# Autodesk Inventor assembly: Full payload assembly mk 2
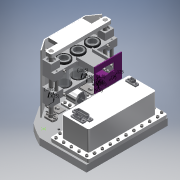
[picture p0: Inventor's stored thumbnail of the model, 180x180]
Saved by Autodesk Inventor 2017 (Build 210142000, 142)
## iProperties
Created: 2016-12-06
Part Number: Full payload assembly mk 2
Document SubType Name: Assembly
Designer: qupec
Mass: 1513.48 g
Surface Area: 2866.97 cm^2
Volume: 582.995 cm^3
Density: 2.59604 g/cm^3
Author: qupec
## Documents named in this file (37)
- D:\UMD Near Space\star\CAD\Mechanical\Full payload assembly mk 2.iam
- D:\UMD Near Space\star\CAD\Mechanical\Subsystems\Slide Rods\Slide rod assembly.iam
- D:\UMD Near Space\star\CAD\Mechanical\Subsystems\Test Tube Rack\Test tube rack.iam
- D:\UMD Near Space\star\CAD\Mechanical\Electonics\STARduino and Pi assembly.iam
- D:\UMD Near Space\star\CAD\Mechanical\Subsystems\Video Capture\Pi Cam and Cable assembly.iam
- D:\UMD Near Space\star\CAD\Mechanical\Electonics\Ribbon Cable Connector-02.ipt
- D:\UMD Near Space\star\CAD\Mechanical\Full payload assembly\AIP\Cable and Harness\Full payload assembly.Harness2.iam
- C:\Users\qupec\Documents\Inventor\Content Center Files\R2017\en-US\U UNC 2603(1)\Unbrako - 4 x 1 - 48 - 1 - Unbrako.ipt
- D:\UMD Near Space\star\CAD\Mechanical\Subsystems\ShakerCAD\ShakerAssembly.iam
- D:\UMD Near Space\star\CAD\Mechanical\Base Plate Mk 2.ipt
- D:\UMD Near Space\star\CAD\Mechanical\Electonics\Electronics Box.ipt
- D:\UMD Near Space\star\CAD\Mechanical\Electonics\Sensor Board.ipt
- D:\UMD Near Space\star\CAD\Mechanical\Electonics\9pin female connector.ipt
- D:\UMD Near Space\star\CAD\Mechanical\Electonics\31pin female connector.ipt
- D:\UMD Near Space\star\CAD\Mechanical\Electonics\15pin female connector.ipt
- C:\Users\qupec\Documents\Inventor\Content Center Files\R2017\en-US\ANSI B18.3(05)\ANSI B18.3 - 4-40 UNC - 0.625(31).ipt
- C:\Users\qupec\Documents\Inventor\Content Center Files\R2017\en-US\ANSI B18.3(05)\ANSI B18.3 - 4-40 UNC - 0.5(31).ipt
- D:\UMD Near Space\star\CAD\Mechanical\Subsystems\Video Capture\LED 5mm.ipt
- C:\Users\qupec\Documents\Inventor\Content Center Files\R2017\en-US\ANSI B18.3(05)\ANSI B18.3 - 4-40 UNC - 0.1875(31).ipt
- D:\UMD Near Space\star\CAD\Mechanical\solar sheild.ipt
- D:\UMD Near Space\star\CAD\Mechanical\Emergency Battery.ipt
- C:\Users\qupec\Documents\Inventor\Content Center Files\R2017\en-US\ANSI B18.3(05)\ANSI B18.3 - 4-40 UNC - 0.75(31).ipt
- D:\UMD Near Space\star\CAD\Mechanical\1556A410_BRACKET.ipt
- D:\UMD Near Space\star\CAD\Mechanical\94518A210_MIL SPEC FLAT-HEAD SOCKET CAP SCREW.ipt
- D:\UMD Near Space\star\CAD\Mechanical\98019A314_MIL SPEC. 300 SERIES SS FLAT WASHER.ipt
- D:\UMD Near Space\star\CAD\Mechanical\Subsystems\Full payload assembly mk 2\AIP\FEA\c3occb59c.fins
- D:\UMD Near Space\star\CAD\Mechanical\Subsystems\Full payload assembly mk 2\AIP\FEA\c3occb5b4.fsat
- D:\UMD Near Space\star\CAD\Mechanical\Subsystems\Full payload assembly mk 2\AIP\FEA\c3occb5b4.ftes
- D:\UMD Near Space\star\CAD\Mechanical\Subsystems\Full payload assembly mk 2\AIP\FEA\c3occb5b4.fwiz
- D:\UMD Near Space\star\CAD\Mechanical\Subsystems\Full payload assembly mk 2\AIP\FEA\c3occb5c0.fins
- D:\UMD Near Space\star\CAD\Mechanical\Subsystems\Full payload assembly mk 2\AIP\FEA\c3occb5c0.fsat
- D:\UMD Near Space\star\CAD\Mechanical\Subsystems\Full payload assembly mk 2\AIP\FEA\c3occb5c0.ftes
- D:\UMD Near Space\star\CAD\Mechanical\Subsystems\Full payload assembly mk 2\AIP\FEA\c3occb5c0.fwiz
- D:\UMD Near Space\star\CAD\Mechanical\Subsystems\Full payload assembly mk 2\AIP\FEA\c3occb60w.fmsh
- D:\UMD Near Space\star\CAD\Mechanical\Subsystems\Full payload assembly mk 2\AIP\FEA\c3occb60x.fres
- D:\UMD Near Space\star\CAD\Mechanical\Subsystems\Full payload assembly mk 2\AIP\FEA\c3occb6sg.fmsh
- D:\UMD Near Space\star\CAD\Mechanical\Subsystems\Full payload assembly mk 2\AIP\FEA\c3occb6sh.fres
## Components (66 placed, 24 different names)
1. Slide rod assembly:1 [sub-assembly] — Mate:119, Mate:120, Mate:121, Mate:278, Mate:280, Mate:282, Mate:284, Mate:286, Mate:288, Mate:290, Mate:292, Mate:294, Mate:296, Flush:47, Mate:382
2. Test tube rack:1 [sub-assembly] — Mate:56, Flush:19, Flush:20, Mate:113, Mate:114, Mate:119, Mate:120, Flush:45
3. Pi Cam and Cable assembly:1 [sub-assembly] — Mate:56, Flush:19, Flush:20, Mate:169, Mate:171, Insert:1, Mate:299, Mate:300, Mate:302, Mate:303, Mate:304
4. Ribbon Cable Connector-02:1 — Mate:80, Flush:24, Flush:25
5. Harness2 [sub-assembly]
6. STARduino and Pi assembly:1 [sub-assembly] — Mate:80, Flush:24, Flush:25, Mate:122, Flush:41, Flush:42, Flush:46
7. ShakerAssembly:1 [sub-assembly] — Mate:113, Mate:114, Flush:26, Mate:123, Angle:2
8. Base Plate Mk 2:1 — Mate:121, Flush:26, Mate:122, Mate:123, Mate:124, Flush:29, Flush:32, Mate:163, Flush:33, Flush:40, Mate:277, Mate:279, Mate:281, Mate:283, Mate:285, Mate:287, Mate:289, Mate:291, Mate:293, Mate:295, Mate:307, Mate:309, Mate:311, Mate:313, Mate:315, Mate:317, Mate:319, Mate:321, Mate:323, Mate:325, Mate:327, Mate:329, Mate:331, Mate:333, Mate:335, Mate:337, Mate:339, Mate:341, Mate:343, Mate:345, Mate:347, Mate:349, Mate:351, Mate:353, Mate:355, Mate:357, Mate:359, Mate:361, Flush:45, Mate:373, Mate:374, Mate:375, Mate:376, Mate:377
9. Sensor Board:1 — Angle:1, Mate:303, Mate:304, Mate:305, Mate:306
10. 31pin female connector:1 — Flush:34, Flush:35, Mate:164
11. 15pin female connector:1 — Mate:165, Flush:43, Flush:44
12. 9pin female connector:1 — Flush:38, Flush:39, Mate:166
13. Electronics Box:1 — Mate:163, Flush:33, Flush:34, Flush:35, Mate:164, Flush:38, Flush:39, Mate:165, Mate:166, Flush:40, Flush:41, Flush:42, Flush:43, Flush:44, Mate:308, Mate:310, Mate:312, Mate:314, Mate:316, Mate:318, Mate:320, Mate:322, Mate:324, Mate:326, Mate:328, Mate:330, Mate:332, Mate:334, Mate:336, Mate:338, Mate:340, Mate:342, Mate:344, Mate:346, Mate:348, Mate:350, Mate:352, Mate:354, Mate:356, Mate:358, Mate:360, Mate:362, Mate:372
14. Hexagon Socket Head Cap Screw - Inch No. 4 - 40 UNC - 1/2:1
15. Hexagon Socket Head Cap Screw - Inch No. 4 - 40 UNC - 1/2:2
16. Unbrako UNC Hex Socket Cap - Inch 4 x 1 - Unbrako:13 — Mate:169, Mate:171
17. Hexagon Socket Head Cap Screw - Inch No. 4 - 40 UNC - 5/8:1 — Mate:277, Mate:278
18. Hexagon Socket Head Cap Screw - Inch No. 4 - 40 UNC - 5/8:2 — Mate:279, Mate:280
19. Hexagon Socket Head Cap Screw - Inch No. 4 - 40 UNC - 5/8:3 — Mate:281, Mate:282
20. Hexagon Socket Head Cap Screw - Inch No. 4 - 40 UNC - 5/8:4 — Mate:283, Mate:284
21. Hexagon Socket Head Cap Screw - Inch No. 4 - 40 UNC - 5/8:5 — Mate:285, Mate:286
22. Hexagon Socket Head Cap Screw - Inch No. 4 - 40 UNC - 5/8:6 — Mate:287, Mate:288
23. Hexagon Socket Head Cap Screw - Inch No. 4 - 40 UNC - 5/8:7 — Mate:289, Mate:290
24. Hexagon Socket Head Cap Screw - Inch No. 4 - 40 UNC - 5/8:8 — Mate:291, Mate:292
25. Hexagon Socket Head Cap Screw - Inch No. 4 - 40 UNC - 5/8:9 — Mate:293, Mate:294
26. Hexagon Socket Head Cap Screw - Inch No. 4 - 40 UNC - 5/8:10 — Mate:295, Mate:296
27. Hexagon Socket Head Cap Screw - Inch No. 4 - 40 UNC - 5/8:11 — Insert:1
28. LED 5mm:1 — Mate:299, Mate:301, Mate:302, Mate:305
29. LED 5mm:2 — Mate:300, Mate:301, Mate:306
30. Hexagon Socket Head Cap Screw - Inch No. 4 - 40 UNC - 3/4:1 — Mate:307, Mate:308
31. Hexagon Socket Head Cap Screw - Inch No. 4 - 40 UNC - 3/4:2 — Mate:309, Mate:310
32. Hexagon Socket Head Cap Screw - Inch No. 4 - 40 UNC - 3/4:3 — Mate:311, Mate:312
33. Hexagon Socket Head Cap Screw - Inch No. 4 - 40 UNC - 3/4:4 — Mate:313, Mate:314
34. Hexagon Socket Head Cap Screw - Inch No. 4 - 40 UNC - 3/4:5 — Mate:315, Mate:316
35. Hexagon Socket Head Cap Screw - Inch No. 4 - 40 UNC - 3/16:6 — Mate:317, Mate:318
36. Hexagon Socket Head Cap Screw - Inch No. 4 - 40 UNC - 3/16:7 — Mate:319, Mate:320
37. Hexagon Socket Head Cap Screw - Inch No. 4 - 40 UNC - 3/16:8 — Mate:321, Mate:322
38. Hexagon Socket Head Cap Screw - Inch No. 4 - 40 UNC - 3/16:9 — Mate:323, Mate:324
39. Hexagon Socket Head Cap Screw - Inch No. 4 - 40 UNC - 3/16:10 — Mate:325, Mate:326
40. Hexagon Socket Head Cap Screw - Inch No. 4 - 40 UNC - 3/16:11 — Mate:327, Mate:328
41. Hexagon Socket Head Cap Screw - Inch No. 4 - 40 UNC - 3/16:12 — Mate:329, Mate:330
42. Hexagon Socket Head Cap Screw - Inch No. 4 - 40 UNC - 3/16:13 — Mate:331, Mate:332
43. Hexagon Socket Head Cap Screw - Inch No. 4 - 40 UNC - 3/16:14 — Mate:333, Mate:334
44. Hexagon Socket Head Cap Screw - Inch No. 4 - 40 UNC - 3/16:15 — Mate:335, Mate:336
45. Hexagon Socket Head Cap Screw - Inch No. 4 - 40 UNC - 3/16:16 — Mate:337, Mate:338
46. Hexagon Socket Head Cap Screw - Inch No. 4 - 40 UNC - 3/16:17 — Mate:339, Mate:340
47. Hexagon Socket Head Cap Screw - Inch No. 4 - 40 UNC - 1/2:3 — Mate:341, Mate:342
48. Hexagon Socket Head Cap Screw - Inch No. 4 - 40 UNC - 3/16:19 — Mate:343, Mate:344
49. Hexagon Socket Head Cap Screw - Inch No. 4 - 40 UNC - 3/16:20 — Mate:345, Mate:346
50. Hexagon Socket Head Cap Screw - Inch No. 4 - 40 UNC - 3/16:21 — Mate:347, Mate:348
51. Hexagon Socket Head Cap Screw - Inch No. 4 - 40 UNC - 3/16:22 — Mate:349, Mate:350
52. Hexagon Socket Head Cap Screw - Inch No. 4 - 40 UNC - 3/16:23 — Mate:351, Mate:352
53. Hexagon Socket Head Cap Screw - Inch No. 4 - 40 UNC - 3/16:24 — Mate:353, Mate:354
54. Hexagon Socket Head Cap Screw - Inch No. 4 - 40 UNC - 3/16:25 — Mate:355, Mate:356
55. Hexagon Socket Head Cap Screw - Inch No. 4 - 40 UNC - 3/16:26 — Mate:357, Mate:358
56. Hexagon Socket Head Cap Screw - Inch No. 4 - 40 UNC - 3/16:27 — Mate:359, Mate:360
57. Hexagon Socket Head Cap Screw - Inch No. 4 - 40 UNC - 3/16:28 — Mate:361, Mate:362
58. solar sheild:1 — Mate:378, Mate:379, Mate:380, Flush:47, Mate:381, Mate:382
59. Emergency Battery:1 — Mate:372, Mate:373, Flush:46
60. 1556A410_BRACKET:1 — Mate:375, Mate:377, Angle:3, Mate:379, Mate:381, Mate:384, Mate:387, Mate:388
61. 1556A410_BRACKET:2 — Mate:374, Mate:376, Angle:2, Angle:3, Mate:378, Mate:380, Mate:383, Mate:386
62. 94518A210_MIL SPEC FLAT-HEAD SOCKET CAP SCREW:1 — Mate:384, Flush:48
63. 94518A210_MIL SPEC FLAT-HEAD SOCKET CAP SCREW:2 — Mate:383, Flush:48, Mate:385
64. 98019A314_MIL SPEC. 300 SERIES SS FLAT WASHER:1
65. 98019A314_MIL SPEC. 300 SERIES SS FLAT WASHER:2 — Mate:385, Mate:386
66. 98019A314_MIL SPEC. 300 SERIES SS FLAT WASHER:3 — Mate:387, Mate:388
## Relationships (146: Mate 121, Flush 21, Angle 3, Insert 1)
- Mate:56: Test tube rack:1 ↔ Pi Cam and Cable assembly:1
- Flush:19: Test tube rack:1 ↔ Pi Cam and Cable assembly:1
- Flush:20: Test tube rack:1 ↔ Pi Cam and Cable assembly:1
- Mate:80: Ribbon Cable Connector-02:1 ↔ STARduino and Pi assembly:1
- Flush:24 (-7 mm): Ribbon Cable Connector-02:1 ↔ STARduino and Pi assembly:1
- Flush:25: Ribbon Cable Connector-02:1 ↔ STARduino and Pi assembly:1
- Mate:113: Test tube rack:1 ↔ ShakerAssembly:1
- Mate:114: Test tube rack:1 ↔ ShakerAssembly:1
- Mate:119: Slide rod assembly:1 ↔ Test tube rack:1
- Mate:120: Slide rod assembly:1 ↔ Test tube rack:1
- Mate:121: Slide rod assembly:1 ↔ Base Plate Mk 2:1
- Flush:26 (6.604 mm): ShakerAssembly:1 ↔ Base Plate Mk 2:1
- Mate:122: STARduino and Pi assembly:1 ↔ Base Plate Mk 2:1
- Mate:123: ShakerAssembly:1 ↔ Base Plate Mk 2:1
- Mate:124: Base Plate Mk 2:1
- Flush:29: Base Plate Mk 2:1
- Flush:32: Base Plate Mk 2:1
- Angle:1 (0 deg): Sensor Board:1
- Mate:163: Base Plate Mk 2:1 ↔ Electronics Box:1
- Flush:33: Base Plate Mk 2:1 ↔ Electronics Box:1
- Flush:34 (12.7 mm): 31pin female connector:1 ↔ Electronics Box:1
- Flush:35 (6.35 mm): 31pin female connector:1 ↔ Electronics Box:1
- Mate:164: 31pin female connector:1 ↔ Electronics Box:1
- Flush:38 (6.35 mm): 9pin female connector:1 ↔ Electronics Box:1
- Flush:39 (-6.35 mm): 9pin female connector:1 ↔ Electronics Box:1
- Mate:165: 15pin female connector:1 ↔ Electronics Box:1
- Mate:166: 9pin female connector:1 ↔ Electronics Box:1
- Flush:40: Base Plate Mk 2:1 ↔ Electronics Box:1
- Flush:41 (3.175 mm): STARduino and Pi assembly:1 ↔ Electronics Box:1
- Flush:42: STARduino and Pi assembly:1 ↔ Electronics Box:1
- Flush:43 (3.81 mm): 15pin female connector:1 ↔ Electronics Box:1
- Flush:44 (12.7 mm): 15pin female connector:1 ↔ Electronics Box:1
- [Mate]: Pi Cam and Cable assembly:1 ↔ Hexagon Socket Head Cap Screw - Inch No. 4 - 40 UNC - 1/2:1
- [Mate]: Pi Cam and Cable assembly:1 ↔ Hexagon Socket Head Cap Screw - Inch No. 4 - 40 UNC - 1/2:2
- Mate:169: Pi Cam and Cable assembly:1 ↔ Unbrako UNC Hex Socket Cap - Inch 4 x 1 - Unbrako:13
- [Mate]: Pi Cam and Cable assembly:1 ↔ Hexagon Socket Head Cap Screw - Inch No. 4 - 40 UNC - 1/2:2
- Mate:171: Pi Cam and Cable assembly:1 ↔ Unbrako UNC Hex Socket Cap - Inch 4 x 1 - Unbrako:13
- [Mate]: Pi Cam and Cable assembly:1 ↔ Hexagon Socket Head Cap Screw - Inch No. 4 - 40 UNC - 1/2:1
- Mate:277: Base Plate Mk 2:1 ↔ Hexagon Socket Head Cap Screw - Inch No. 4 - 40 UNC - 5/8:1
- Mate:278: Slide rod assembly:1 ↔ Hexagon Socket Head Cap Screw - Inch No. 4 - 40 UNC - 5/8:1
- Mate:279: Base Plate Mk 2:1 ↔ Hexagon Socket Head Cap Screw - Inch No. 4 - 40 UNC - 5/8:2
- Mate:280: Slide rod assembly:1 ↔ Hexagon Socket Head Cap Screw - Inch No. 4 - 40 UNC - 5/8:2
- Mate:281: Base Plate Mk 2:1 ↔ Hexagon Socket Head Cap Screw - Inch No. 4 - 40 UNC - 5/8:3
- Mate:282: Slide rod assembly:1 ↔ Hexagon Socket Head Cap Screw - Inch No. 4 - 40 UNC - 5/8:3
- Mate:283: Base Plate Mk 2:1 ↔ Hexagon Socket Head Cap Screw - Inch No. 4 - 40 UNC - 5/8:4
- Mate:284: Slide rod assembly:1 ↔ Hexagon Socket Head Cap Screw - Inch No. 4 - 40 UNC - 5/8:4
- Mate:285: Base Plate Mk 2:1 ↔ Hexagon Socket Head Cap Screw - Inch No. 4 - 40 UNC - 5/8:5
- Mate:286: Slide rod assembly:1 ↔ Hexagon Socket Head Cap Screw - Inch No. 4 - 40 UNC - 5/8:5
- Mate:287: Base Plate Mk 2:1 ↔ Hexagon Socket Head Cap Screw - Inch No. 4 - 40 UNC - 5/8:6
- Mate:288: Slide rod assembly:1 ↔ Hexagon Socket Head Cap Screw - Inch No. 4 - 40 UNC - 5/8:6
- Mate:289: Base Plate Mk 2:1 ↔ Hexagon Socket Head Cap Screw - Inch No. 4 - 40 UNC - 5/8:7
- Mate:290: Slide rod assembly:1 ↔ Hexagon Socket Head Cap Screw - Inch No. 4 - 40 UNC - 5/8:7
- Mate:291: Base Plate Mk 2:1 ↔ Hexagon Socket Head Cap Screw - Inch No. 4 - 40 UNC - 5/8:8
- Mate:292: Slide rod assembly:1 ↔ Hexagon Socket Head Cap Screw - Inch No. 4 - 40 UNC - 5/8:8
- Mate:293: Base Plate Mk 2:1 ↔ Hexagon Socket Head Cap Screw - Inch No. 4 - 40 UNC - 5/8:9
- Mate:294: Slide rod assembly:1 ↔ Hexagon Socket Head Cap Screw - Inch No. 4 - 40 UNC - 5/8:9
- Mate:295: Base Plate Mk 2:1 ↔ Hexagon Socket Head Cap Screw - Inch No. 4 - 40 UNC - 5/8:10
- Mate:296: Slide rod assembly:1 ↔ Hexagon Socket Head Cap Screw - Inch No. 4 - 40 UNC - 5/8:10
- Insert:1: Pi Cam and Cable assembly:1 ↔ Hexagon Socket Head Cap Screw - Inch No. 4 - 40 UNC - 5/8:11
- Mate:299: Pi Cam and Cable assembly:1 ↔ LED 5mm:1
- Mate:300: Pi Cam and Cable assembly:1 ↔ LED 5mm:2
- Mate:301: LED 5mm:1 ↔ LED 5mm:2
- Mate:302: Pi Cam and Cable assembly:1 ↔ LED 5mm:1
- Mate:303: Pi Cam and Cable assembly:1 ↔ Sensor Board:1
- Mate:304: Pi Cam and Cable assembly:1 ↔ Sensor Board:1
- Mate:305: Sensor Board:1 ↔ LED 5mm:1
- Mate:306: Sensor Board:1 ↔ LED 5mm:2
- Mate:307: Base Plate Mk 2:1 ↔ Hexagon Socket Head Cap Screw - Inch No. 4 - 40 UNC - 3/4:1
- Mate:308: Electronics Box:1 ↔ Hexagon Socket Head Cap Screw - Inch No. 4 - 40 UNC - 3/4:1
- Mate:309: Base Plate Mk 2:1 ↔ Hexagon Socket Head Cap Screw - Inch No. 4 - 40 UNC - 3/4:2
- Mate:310: Electronics Box:1 ↔ Hexagon Socket Head Cap Screw - Inch No. 4 - 40 UNC - 3/4:2
- Mate:311: Base Plate Mk 2:1 ↔ Hexagon Socket Head Cap Screw - Inch No. 4 - 40 UNC - 3/4:3
- Mate:312: Electronics Box:1 ↔ Hexagon Socket Head Cap Screw - Inch No. 4 - 40 UNC - 3/4:3
- Mate:313: Base Plate Mk 2:1 ↔ Hexagon Socket Head Cap Screw - Inch No. 4 - 40 UNC - 3/4:4
- Mate:314: Electronics Box:1 ↔ Hexagon Socket Head Cap Screw - Inch No. 4 - 40 UNC - 3/4:4
- Mate:315: Base Plate Mk 2:1 ↔ Hexagon Socket Head Cap Screw - Inch No. 4 - 40 UNC - 3/4:5
- Mate:316: Electronics Box:1 ↔ Hexagon Socket Head Cap Screw - Inch No. 4 - 40 UNC - 3/4:5
- Mate:317: Base Plate Mk 2:1 ↔ Hexagon Socket Head Cap Screw - Inch No. 4 - 40 UNC - 3/16:6
- Mate:318: Electronics Box:1 ↔ Hexagon Socket Head Cap Screw - Inch No. 4 - 40 UNC - 3/16:6
- Mate:319: Base Plate Mk 2:1 ↔ Hexagon Socket Head Cap Screw - Inch No. 4 - 40 UNC - 3/16:7
- Mate:320: Electronics Box:1 ↔ Hexagon Socket Head Cap Screw - Inch No. 4 - 40 UNC - 3/16:7
- Mate:321: Base Plate Mk 2:1 ↔ Hexagon Socket Head Cap Screw - Inch No. 4 - 40 UNC - 3/16:8
- Mate:322: Electronics Box:1 ↔ Hexagon Socket Head Cap Screw - Inch No. 4 - 40 UNC - 3/16:8
- Mate:323: Base Plate Mk 2:1 ↔ Hexagon Socket Head Cap Screw - Inch No. 4 - 40 UNC - 3/16:9
- Mate:324: Electronics Box:1 ↔ Hexagon Socket Head Cap Screw - Inch No. 4 - 40 UNC - 3/16:9
- Mate:325: Base Plate Mk 2:1 ↔ Hexagon Socket Head Cap Screw - Inch No. 4 - 40 UNC - 3/16:10
- Mate:326: Electronics Box:1 ↔ Hexagon Socket Head Cap Screw - Inch No. 4 - 40 UNC - 3/16:10
- Mate:327: Base Plate Mk 2:1 ↔ Hexagon Socket Head Cap Screw - Inch No. 4 - 40 UNC - 3/16:11
- Mate:328: Electronics Box:1 ↔ Hexagon Socket Head Cap Screw - Inch No. 4 - 40 UNC - 3/16:11
- Mate:329: Base Plate Mk 2:1 ↔ Hexagon Socket Head Cap Screw - Inch No. 4 - 40 UNC - 3/16:12
- Mate:330: Electronics Box:1 ↔ Hexagon Socket Head Cap Screw - Inch No. 4 - 40 UNC - 3/16:12
- Mate:331: Base Plate Mk 2:1 ↔ Hexagon Socket Head Cap Screw - Inch No. 4 - 40 UNC - 3/16:13
- Mate:332: Electronics Box:1 ↔ Hexagon Socket Head Cap Screw - Inch No. 4 - 40 UNC - 3/16:13
- Mate:333: Base Plate Mk 2:1 ↔ Hexagon Socket Head Cap Screw - Inch No. 4 - 40 UNC - 3/16:14
- Mate:334: Electronics Box:1 ↔ Hexagon Socket Head Cap Screw - Inch No. 4 - 40 UNC - 3/16:14
- Mate:335: Base Plate Mk 2:1 ↔ Hexagon Socket Head Cap Screw - Inch No. 4 - 40 UNC - 3/16:15
- Mate:336: Electronics Box:1 ↔ Hexagon Socket Head Cap Screw - Inch No. 4 - 40 UNC - 3/16:15
- Mate:337: Base Plate Mk 2:1 ↔ Hexagon Socket Head Cap Screw - Inch No. 4 - 40 UNC - 3/16:16
- Mate:338: Electronics Box:1 ↔ Hexagon Socket Head Cap Screw - Inch No. 4 - 40 UNC - 3/16:16
- Mate:339: Base Plate Mk 2:1 ↔ Hexagon Socket Head Cap Screw - Inch No. 4 - 40 UNC - 3/16:17
- Mate:340: Electronics Box:1 ↔ Hexagon Socket Head Cap Screw - Inch No. 4 - 40 UNC - 3/16:17
- Mate:341: Base Plate Mk 2:1 ↔ Hexagon Socket Head Cap Screw - Inch No. 4 - 40 UNC - 1/2:3
- Mate:342: Electronics Box:1 ↔ Hexagon Socket Head Cap Screw - Inch No. 4 - 40 UNC - 1/2:3
- Mate:343: Base Plate Mk 2:1 ↔ Hexagon Socket Head Cap Screw - Inch No. 4 - 40 UNC - 3/16:19
- Mate:344: Electronics Box:1 ↔ Hexagon Socket Head Cap Screw - Inch No. 4 - 40 UNC - 3/16:19
- Mate:345: Base Plate Mk 2:1 ↔ Hexagon Socket Head Cap Screw - Inch No. 4 - 40 UNC - 3/16:20
- Mate:346: Electronics Box:1 ↔ Hexagon Socket Head Cap Screw - Inch No. 4 - 40 UNC - 3/16:20
- Mate:347: Base Plate Mk 2:1 ↔ Hexagon Socket Head Cap Screw - Inch No. 4 - 40 UNC - 3/16:21
- Mate:348: Electronics Box:1 ↔ Hexagon Socket Head Cap Screw - Inch No. 4 - 40 UNC - 3/16:21
- Mate:349: Base Plate Mk 2:1 ↔ Hexagon Socket Head Cap Screw - Inch No. 4 - 40 UNC - 3/16:22
- Mate:350: Electronics Box:1 ↔ Hexagon Socket Head Cap Screw - Inch No. 4 - 40 UNC - 3/16:22
- Mate:351: Base Plate Mk 2:1 ↔ Hexagon Socket Head Cap Screw - Inch No. 4 - 40 UNC - 3/16:23
- Mate:352: Electronics Box:1 ↔ Hexagon Socket Head Cap Screw - Inch No. 4 - 40 UNC - 3/16:23
- Mate:353: Base Plate Mk 2:1 ↔ Hexagon Socket Head Cap Screw - Inch No. 4 - 40 UNC - 3/16:24
- Mate:354: Electronics Box:1 ↔ Hexagon Socket Head Cap Screw - Inch No. 4 - 40 UNC - 3/16:24
- Mate:355: Base Plate Mk 2:1 ↔ Hexagon Socket Head Cap Screw - Inch No. 4 - 40 UNC - 3/16:25
- Mate:356: Electronics Box:1 ↔ Hexagon Socket Head Cap Screw - Inch No. 4 - 40 UNC - 3/16:25
- Mate:357: Base Plate Mk 2:1 ↔ Hexagon Socket Head Cap Screw - Inch No. 4 - 40 UNC - 3/16:26
- Mate:358: Electronics Box:1 ↔ Hexagon Socket Head Cap Screw - Inch No. 4 - 40 UNC - 3/16:26
- Mate:359: Base Plate Mk 2:1 ↔ Hexagon Socket Head Cap Screw - Inch No. 4 - 40 UNC - 3/16:27
- Mate:360: Electronics Box:1 ↔ Hexagon Socket Head Cap Screw - Inch No. 4 - 40 UNC - 3/16:27
- Mate:361: Base Plate Mk 2:1 ↔ Hexagon Socket Head Cap Screw - Inch No. 4 - 40 UNC - 3/16:28
- Mate:362: Electronics Box:1 ↔ Hexagon Socket Head Cap Screw - Inch No. 4 - 40 UNC - 3/16:28
- Flush:45: Test tube rack:1 ↔ Base Plate Mk 2:1
- Mate:372: Electronics Box:1 ↔ Emergency Battery:1
- Mate:373: Base Plate Mk 2:1 ↔ Emergency Battery:1
- Flush:46: STARduino and Pi assembly:1 ↔ Emergency Battery:1
- Mate:374: Base Plate Mk 2:1 ↔ 1556A410_BRACKET:2
- Mate:375: Base Plate Mk 2:1 ↔ 1556A410_BRACKET:1
- Mate:376: Base Plate Mk 2:1 ↔ 1556A410_BRACKET:2
- Mate:377: Base Plate Mk 2:1 ↔ 1556A410_BRACKET:1
- Angle:2 (0 deg): ShakerAssembly:1 ↔ 1556A410_BRACKET:2
- Angle:3 (0 deg): 1556A410_BRACKET:1 ↔ 1556A410_BRACKET:2
- Mate:378: solar sheild:1 ↔ 1556A410_BRACKET:2
- Mate:379: solar sheild:1 ↔ 1556A410_BRACKET:1
- Mate:380: solar sheild:1 ↔ 1556A410_BRACKET:2
- Flush:47: Slide rod assembly:1 ↔ solar sheild:1
- Mate:381: solar sheild:1 ↔ 1556A410_BRACKET:1
- Mate:382: Slide rod assembly:1 ↔ solar sheild:1
- Mate:383: 1556A410_BRACKET:2 ↔ 94518A210_MIL SPEC FLAT-HEAD SOCKET CAP SCREW:2
- Mate:384: 1556A410_BRACKET:1 ↔ 94518A210_MIL SPEC FLAT-HEAD SOCKET CAP SCREW:1
- Flush:48: 94518A210_MIL SPEC FLAT-HEAD SOCKET CAP SCREW:1 ↔ 94518A210_MIL SPEC FLAT-HEAD SOCKET CAP SCREW:2
- Mate:385: 94518A210_MIL SPEC FLAT-HEAD SOCKET CAP SCREW:2 ↔ 98019A314_MIL SPEC. 300 SERIES SS FLAT WASHER:2
- Mate:386: 1556A410_BRACKET:2 ↔ 98019A314_MIL SPEC. 300 SERIES SS FLAT WASHER:2
- Mate:387: 1556A410_BRACKET:1 ↔ 98019A314_MIL SPEC. 300 SERIES SS FLAT WASHER:3
- Mate:388: 1556A410_BRACKET:1 ↔ 98019A314_MIL SPEC. 300 SERIES SS FLAT WASHER:3
## Named parameters: sa_3 = 0, sa_4 = 29260.8, sa_5 = 0, sa_6 = 6894.76
note: some values were not read from the file. Shown as the stored number, unit unknown: "sa_3", "sa_4", "sa_5", "sa_6".
